# Autodesk Inventor assembly: panelB_onFrame
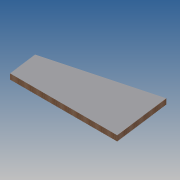
[picture p0: Inventor's stored thumbnail of the model, 180x180]
Saved by Autodesk Inventor 2014 SP1 (Build 180222100, 222)
## iProperties
Created: 2015-02-13
Part Number: panelB_onFrame
Document SubType Name: Assembly
Designer: Dave
Author: Dave
## Documents named in this file (3)
- C:\Users\Dave\Desktop\hera-cad\surface\panelB_onFrame.iam
- C:\Users\Dave\Desktop\hera-cad\surface\panelBflat.ipt
- C:\Users\Dave\Desktop\hera-cad\surface\panelBframe.ipt
## Components (2 placed, 2 different names)
1. panelBflat:1 — Mate:1, Flush:1, Flush:2
2. panelBframe:1 — Mate:1, Flush:1, Flush:2
## Relationships (3: Flush 2, Mate 1)
- Mate:1: panelBflat:1 ↔ panelBframe:1
- Flush:1: panelBflat:1 ↔ panelBframe:1
- Flush:2: panelBflat:1 ↔ panelBframe:1
